# Autodesk Inventor assembly: Shoulder_nema24_v2
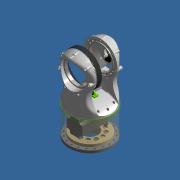
[picture p0: Inventor's stored thumbnail of the model, 180x180]
Saved by Autodesk Inventor 2016 (Build 200138000, 138)
## iProperties
Created: 2015-01-06
Part Number: Shoulder_nema24_v2
Document SubType Name: Assembly
Designer: 4ndreas
Mass: 6291.08 g
Surface Area: 5886.11 cm^2
Volume: 2540.03 cm^3
Density: 2.47677 g/cm^3
Author: 4ndreas
## Documents named in this file (20)
- C:\Users\4ndreas\Documents\Inventor\RobotARM v2\v4\Shoulder_nema24_v2.iam
- C:\Users\4ndreas\Documents\Inventor\RobotARM v2\v2\BaseJoint\Konstruktions-Assistent\Übertragung des Zahnriemens1.iam
- C:\Users\4ndreas\Documents\Inventor\Content Center Files\R2014\de-DE\DIN 125-1  A\DIN 125 - A 4,3.ipt
- C:\Users\4ndreas\Documents\Inventor\Content Center Files\R2014\de-DE\DIN BEARING(1)\DIN 625 SKF - SKF 624.ipt
- C:\Users\4ndreas\Documents\Inventor\RobotARM v2\v3\Shoulder_spanner.ipt
- C:\Users\4ndreas\Documents\Inventor\Content Center Files\R2014\de-DE\DIN 934\DIN 934 - M4 x 0,7.ipt
- C:\Users\4ndreas\Documents\Inventor\RobotARM v2\v2\encoder.iam
- C:\Users\4ndreas\Documents\Inventor\Content Center Files\R2014\de-DE\DIN 912\DIN 912 - M4 x 0,7 x 35 x 20.ipt
- C:\Users\4ndreas\Documents\Inventor\RobotARM v2\v4\Shoulder_stepper\Konstruktions-Assistent\Übertragung des Zahnriemens1.iam
- C:\Users\4ndreas\Documents\Inventor\Content Center Files\R2014\de-DE\DIN BEARING(1)\DIN 625 SKF - SKF 61818.ipt
- C:\Users\4ndreas\Documents\Inventor\RobotARM v2\v4\Shoulder_basis_N24.ipt
- C:\Users\4ndreas\Documents\Inventor\RobotARM v2\v4\CoverBase.ipt
- C:\Users\4ndreas\Documents\Inventor\RobotARM v2\v4\Shoulder_nema24_v2\Konstruktions-Assistent\Welle1.iam
- C:\Users\4ndreas\Documents\Inventor\RobotARM v2\v4\Nema24_100.ipt
- C:\Users\4ndreas\Documents\Inventor\Content Center Files\R2014\de-DE\DIN BEARING(1)\DIN 625 SKF - SKF 608.ipt
- C:\Users\4ndreas\Documents\Inventor\RobotARM v2\v4\PRT_02_60_AL_2.iam
- C:\Users\4ndreas\Documents\Inventor\RobotARM v2\v4\16224800.ipt
- C:\Users\4ndreas\Documents\Inventor\Content Center Files\R2014\de-DE\DIN 125-1  A\DIN 125 - A 8,4.ipt
- C:\Users\4ndreas\Documents\Inventor\RobotARM v2\v4\LagerKlemme.ipt
- C:\Users\4ndreas\Documents\Inventor\RobotARM v2\v4\16221600.ipt
## Components (35 placed, 18 different names)
1. Übertragung des Zahnriemens:1 [sub-assembly] — Passend:1, Passend:12, Passend:49, Passend:69, Passend:94, Passend:95, Passend:138, Fluchtend:18, Passend:147, Tangential:1, Passend:173
2. DIN 912 - ersetzt durch DIN EN ISO 4762 M4 x 35:2 — Passend:70, Passend:71, Passend:77, Passend:78, Passend:97, Passend:176
3. DIN 912 - ersetzt durch DIN EN ISO 4762 M4 x 35:1 — Passend:69, Passend:73, Passend:74, Passend:82, Passend:99, Passend:179
4. DIN 125-1 A A 4,3:1 — Passend:70, Passend:71, Fluchtend:9
5. DIN 125-1 A A 4,3:2 — Passend:73, Passend:74, Fluchtend:9
6. DIN 625 SKF SKF 624:1 — Passend:78, Passend:178
7. DIN 625 SKF SKF 624:2 — Passend:77, Tangential:1, Passend:177
8. DIN 625 SKF SKF 624:3 — Passend:80, Passend:82, Passend:181
9. DIN 625 SKF SKF 624:4 — Passend:80, Passend:180
10. DIN 125-1 A A 4,3:3
11. DIN 125-1 A A 4,3:4
12. DIN 125-1 A A 4,3:5
13. DIN 125-1 A A 4,3:6
14. Shoulder_spanner:1 — Passend:94, Passend:95, Passend:96, Passend:98, Passend:100, Passend:101, Passend:102
15. DIN 934 - ersetzt durch DIN EN 24032/28673/28674 M4:1 — Passend:99, Passend:100, Passend:101
16. DIN 934 - ersetzt durch DIN EN 24032/28673/28674 M4:2 — Passend:97, Passend:98, Passend:102
17. encoder:2 [sub-assembly] — Passend:116, Passend:162, Passend:163
18. Übertragung des Zahnriemens:2 [sub-assembly] — Passend:130
19. Nema24_100:1 — Passend:130, Winkel:10, Passend:174, Passend:175
20. DIN 625 SKF SKF 61818:1 — Passend:138, Passend:142
21. Shoulder_basis_N24:1 — Passend:139, Fluchtend:14, Passend:140, Fluchtend:16, Passend:142, Passend:143, Passend:144, Fluchtend:17, Passend:162, Passend:163, Passend:164, Passend:169, Fluchtend:19
22. CoverBase:1 — Passend:143, Passend:156, Passend:157, Passend:164
23. DIN 625 SKF SKF 61818:2 — Passend:144, Fluchtend:17
24. Welle:1 [sub-assembly] — Fluchtend:18, Passend:147, Passend:153, Passend:154, Passend:155, Passend:165, Passend:166
25. DIN 625 SKF SKF 608:1 — Passend:153, Passend:167, Passend:169
26. DIN 625 SKF SKF 608:3 — Passend:154, Passend:170, Passend:171
27. DIN 625 SKF SKF 608:4 — Passend:155
28. PRT_02_60_AL_2:1 [sub-assembly] — Passend:156, Passend:157
29. 16224800:1 — Passend:165, Passend:172
30. DIN 125-1 A A 8,4:1 — Passend:166, Passend:167, Passend:172
31. DIN 125-1 A A 8,4:2 — Passend:170, Passend:171, Passend:173
32. LagerKlemme:1 — Fluchtend:19
33. 16221600:1 — Passend:174, Passend:175
34. DIN 625 SKF SKF 624:5 — Passend:176, Passend:177, Passend:178
35. DIN 625 SKF SKF 624:6 — Passend:179, Passend:180, Passend:181
## Relationships (75: Mate 65, Flush 8, Angle 1, Tangent 1)
- Passend:1 [Mate]: Übertragung des Zahnriemens:1
- Passend:4 [Mate]
- Passend:12 [Mate]: Übertragung des Zahnriemens:1
- Passend:49 [Mate]: Übertragung des Zahnriemens:1
- Passend:62 [Mate]
- Passend:63 [Mate]
- Passend:69 [Mate]: Übertragung des Zahnriemens:1 ↔ DIN 912 - ersetzt durch DIN EN ISO 4762 M4 x 35:1
- Passend:70 [Mate]: DIN 912 - ersetzt durch DIN EN ISO 4762 M4 x 35:2 ↔ DIN 125-1 A A 4,3:1
- Passend:71 [Mate]: DIN 912 - ersetzt durch DIN EN ISO 4762 M4 x 35:2 ↔ DIN 125-1 A A 4,3:1
- Passend:73 [Mate]: DIN 912 - ersetzt durch DIN EN ISO 4762 M4 x 35:1 ↔ DIN 125-1 A A 4,3:2
- Passend:74 [Mate]: DIN 912 - ersetzt durch DIN EN ISO 4762 M4 x 35:1 ↔ DIN 125-1 A A 4,3:2
- Passend:77 [Mate]: DIN 912 - ersetzt durch DIN EN ISO 4762 M4 x 35:2 ↔ DIN 625 SKF SKF 624:2
- Passend:78 [Mate]: DIN 912 - ersetzt durch DIN EN ISO 4762 M4 x 35:2 ↔ DIN 625 SKF SKF 624:1
- Passend:80 [Mate]: DIN 625 SKF SKF 624:3 ↔ DIN 625 SKF SKF 624:4
- Passend:82 [Mate]: DIN 912 - ersetzt durch DIN EN ISO 4762 M4 x 35:1 ↔ DIN 625 SKF SKF 624:3
- [Mate]: DIN 912 - ersetzt durch DIN EN ISO 4762 M4 x 35:1 ↔ DIN 125-1 A A 4,3:4
- [Mate]: DIN 625 SKF SKF 624:3 ↔ DIN 125-1 A A 4,3:4
- [Mate]: DIN 912 - ersetzt durch DIN EN ISO 4762 M4 x 35:1 ↔ DIN 125-1 A A 4,3:5
- [Mate]: DIN 625 SKF SKF 624:4 ↔ DIN 125-1 A A 4,3:5
- [Mate]: DIN 912 - ersetzt durch DIN EN ISO 4762 M4 x 35:2 ↔ DIN 125-1 A A 4,3:3
- [Mate]: DIN 912 - ersetzt durch DIN EN ISO 4762 M4 x 35:2 ↔ DIN 125-1 A A 4,3:6
- [Mate]: DIN 625 SKF SKF 624:2 ↔ DIN 125-1 A A 4,3:6
- [Mate]: DIN 625 SKF SKF 624:1 ↔ DIN 125-1 A A 4,3:3
- Passend:94 [Mate]: Übertragung des Zahnriemens:1 ↔ Shoulder_spanner:1
- Passend:95 [Mate]: Übertragung des Zahnriemens:1 ↔ Shoulder_spanner:1
- Passend:96 [Mate]: Shoulder_spanner:1
- Passend:97 [Mate]: DIN 912 - ersetzt durch DIN EN ISO 4762 M4 x 35:2 ↔ DIN 934 - ersetzt durch DIN EN 24032/28673/28674 M4:2
- Passend:98 [Mate]: Shoulder_spanner:1 ↔ DIN 934 - ersetzt durch DIN EN 24032/28673/28674 M4:2
- Passend:99 [Mate]: DIN 912 - ersetzt durch DIN EN ISO 4762 M4 x 35:1 ↔ DIN 934 - ersetzt durch DIN EN 24032/28673/28674 M4:1
- Passend:100 [Mate]: Shoulder_spanner:1 ↔ DIN 934 - ersetzt durch DIN EN 24032/28673/28674 M4:1
- Passend:101 [Mate]: Shoulder_spanner:1 ↔ DIN 934 - ersetzt durch DIN EN 24032/28673/28674 M4:1
- Passend:102 [Mate]: Shoulder_spanner:1 ↔ DIN 934 - ersetzt durch DIN EN 24032/28673/28674 M4:2
- Fluchtend:9 [Flush]: DIN 125-1 A A 4,3:1 ↔ DIN 125-1 A A 4,3:2
- Passend:116 [Mate]: encoder:2
- Fluchtend:12 [Flush] (43 mm)
- Fluchtend:13 [Flush] (20 mm)
- Passend:130 [Mate]: Übertragung des Zahnriemens:2 ↔ Nema24_100:1
- Winkel:10 [Angle] (0 deg): Nema24_100:1
- Passend:138 [Mate]: Übertragung des Zahnriemens:1 ↔ DIN 625 SKF SKF 61818:1
- Passend:139 [Mate]: Shoulder_basis_N24:1
- Fluchtend:14 [Flush]: Shoulder_basis_N24:1
- Passend:140 [Mate]: Shoulder_basis_N24:1
- Fluchtend:16 [Flush]: Shoulder_basis_N24:1
- Passend:142 [Mate]: DIN 625 SKF SKF 61818:1 ↔ Shoulder_basis_N24:1
- Passend:143 [Mate]: Shoulder_basis_N24:1 ↔ CoverBase:1
- Passend:144 [Mate]: Shoulder_basis_N24:1 ↔ DIN 625 SKF SKF 61818:2
- Fluchtend:17 [Flush]: Shoulder_basis_N24:1 ↔ DIN 625 SKF SKF 61818:2
- Fluchtend:18 [Flush] (-10 mm): Übertragung des Zahnriemens:1 ↔ Welle:1
- Passend:147 [Mate]: Übertragung des Zahnriemens:1 ↔ Welle:1
- Passend:153 [Mate]: Welle:1 ↔ DIN 625 SKF SKF 608:1
- Passend:154 [Mate]: Welle:1 ↔ DIN 625 SKF SKF 608:3
- Passend:155 [Mate]: Welle:1 ↔ DIN 625 SKF SKF 608:4
- Passend:156 [Mate]: CoverBase:1 ↔ PRT_02_60_AL_2:1
- Passend:157 [Mate]: CoverBase:1 ↔ PRT_02_60_AL_2:1
- Passend:162 [Mate]: encoder:2 ↔ Shoulder_basis_N24:1
- Passend:163 [Mate]: encoder:2 ↔ Shoulder_basis_N24:1
- Passend:164 [Mate]: Shoulder_basis_N24:1 ↔ CoverBase:1
- Passend:165 [Mate]: Welle:1 ↔ 16224800:1
- Passend:166 [Mate]: Welle:1 ↔ DIN 125-1 A A 8,4:1
- Passend:167 [Mate]: DIN 625 SKF SKF 608:1 ↔ DIN 125-1 A A 8,4:1
- Passend:169 [Mate]: Shoulder_basis_N24:1 ↔ DIN 625 SKF SKF 608:1
- Passend:170 [Mate]: DIN 625 SKF SKF 608:3 ↔ DIN 125-1 A A 8,4:2
- Passend:171 [Mate]: DIN 625 SKF SKF 608:3 ↔ DIN 125-1 A A 8,4:2
- Tangential:1: Übertragung des Zahnriemens:1 ↔ DIN 625 SKF SKF 624:2
- Passend:172 [Mate]: 16224800:1 ↔ DIN 125-1 A A 8,4:1
- Passend:173 [Mate] (0.5 mm): Übertragung des Zahnriemens:1 ↔ DIN 125-1 A A 8,4:2
- Fluchtend:19 [Flush]: Shoulder_basis_N24:1 ↔ LagerKlemme:1
- Passend:174 [Mate]: Nema24_100:1 ↔ 16221600:1
- Passend:175 [Mate] (0.5 mm): Nema24_100:1 ↔ 16221600:1
- Passend:176 [Mate]: DIN 912 - ersetzt durch DIN EN ISO 4762 M4 x 35:2 ↔ DIN 625 SKF SKF 624:5
- Passend:177 [Mate]: DIN 625 SKF SKF 624:2 ↔ DIN 625 SKF SKF 624:5
- Passend:178 [Mate]: DIN 625 SKF SKF 624:1 ↔ DIN 625 SKF SKF 624:5
- Passend:179 [Mate]: DIN 912 - ersetzt durch DIN EN ISO 4762 M4 x 35:1 ↔ DIN 625 SKF SKF 624:6
- Passend:180 [Mate]: DIN 625 SKF SKF 624:4 ↔ DIN 625 SKF SKF 624:6
- Passend:181 [Mate]: DIN 625 SKF SKF 624:3 ↔ DIN 625 SKF SKF 624:6
